# Autodesk Inventor assembly: Нога левая в сборе_MIR
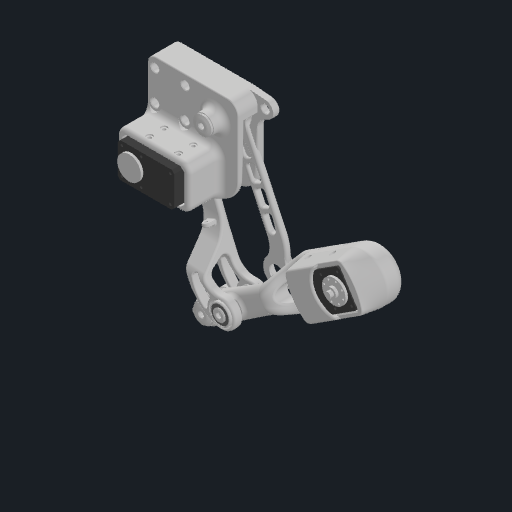
[picture p0: Inventor's stored thumbnail of the model, 512x512]
Saved by Autodesk Inventor 2025 (Build 290162010, 162A)
## iProperties
Created: 2024-06-21
Part Number: Нога левая в сборе_MIR
Document SubType Name: Assembly
Designer: Edward_Higgins
Author: Edward_Higgins
## Documents named in this file (16)
- D:\Users\Edward_Higgins\Desktop\ZAVOD\Робот Сколково\Нога левая в сборе_MIR.iam
- D:\Users\Edward_Higgins\Desktop\ZAVOD\Робот Сколково\Тяга передняя_MIR.ipt
- D:\Users\Edward_Higgins\Desktop\ZAVOD\Робот Сколково\DYNAMIXEL XM430-W350.ipt
- D:\Users\Edward_Higgins\Desktop\ZAVOD\Робот Сколково\Корпус ноги_MIR.ipt
- D:\Users\Edward_Higgins\Desktop\ZAVOD\Робот Сколково\Голень в сборе.iam
- D:\Users\Edward_Higgins\Desktop\ZAVOD\Робот Сколково\Тяга задняя 2_MIR.ipt
- D:\Users\Edward_Higgins\Desktop\ZAVOD\Робот Сколково\Подшипник.ipt
- D:\Users\Edward_Higgins\Desktop\ZAVOD\Робот Сколково\Стопорная шайба.ipt
- D:\Users\Edward_Higgins\Desktop\ZAVOD\Робот Сколково\Шайба.ipt
- D:\Users\Edward_Higgins\Desktop\ZAVOD\Робот Сколково\Ось односторонняя.ipt
- D:\Users\Edward_Higgins\Desktop\ZAVOD\Робот Сколково\Нога левая в сборе\AIP\FEA\ew5x1yt5s.fins
- D:\Users\Edward_Higgins\Desktop\ZAVOD\Робот Сколково\Нога левая в сборе\AIP\FEA\ew5x1yt5s.fsat
- D:\Users\Edward_Higgins\Desktop\ZAVOD\Робот Сколково\Нога левая в сборе\AIP\FEA\ew5x1yt5s.ftes
- D:\Users\Edward_Higgins\Desktop\ZAVOD\Робот Сколково\Нога левая в сборе\AIP\FEA\ew5x1yt5s.fwiz
- D:\Users\Edward_Higgins\Desktop\ZAVOD\Робот Сколково\Нога левая в сборе\AIP\FEA\ew5x1yt6o.fmsh
- D:\Users\Edward_Higgins\Desktop\ZAVOD\Робот Сколково\Нога левая в сборе\AIP\FEA\ew5x1yt6p.fres
## Components (9 placed, 9 different names)
1. Тяга передняя левая:1 — Совмещение:84, Совмещение:85, Совмещение:28, Совмещение:29
2. DYNAMIXEL XM430-W350:1 — Совмещение:84, Совмещение:83, Угол:1, Совмещение:29, Совмещение:30
3. Корпус ноги левый:1 — Совмещение:83, Угол:1, Совмещение:15, Совмещение:14, Совмещение:98, Совмещение:21, Совмещение:30
4. Голень в сборе:1 [sub-assembly] — Совмещение:85, Совмещение:27, Совмещение:28, Совмещение:32
5. Тяга задняя левая:1 — Совмещение:22, Совмещение:23, Совмещение:24, Совмещение:27, Совмещение:32, Совмещение:33
6. Подшипник:1 — Совмещение:93, Совмещение:25, Совмещение:26, Совмещение:33
7. Шайба:1 — Совмещение:23, Совмещение:24
8. Ось односторонняя:1 — Совмещение:98, Совмещение:93, Совмещение:21, Совмещение:22
9. Стопорная шайба:2 — Совмещение:25, Совмещение:26
## Relationships (20: Mate 19, Angle 1)
- Совмещение:84 [Mate]: Тяга передняя левая:1 ↔ DYNAMIXEL XM430-W350:1
- Совмещение:83 [Mate]: DYNAMIXEL XM430-W350:1 ↔ Корпус ноги левый:1
- Угол:1 [Angle] (0 deg): DYNAMIXEL XM430-W350:1 ↔ Корпус ноги левый:1
- Совмещение:15 [Mate]: Корпус ноги левый:1
- Совмещение:14 [Mate]: Корпус ноги левый:1
- Совмещение:85 [Mate]: Тяга передняя левая:1 ↔ Голень в сборе:1
- Совмещение:98 [Mate]: Корпус ноги левый:1 ↔ Ось односторонняя:1
- Совмещение:93 [Mate]: Подшипник:1 ↔ Ось односторонняя:1
- Совмещение:21 [Mate]: Корпус ноги левый:1 ↔ Ось односторонняя:1
- Совмещение:22 [Mate]: Тяга задняя левая:1 ↔ Ось односторонняя:1
- Совмещение:23 [Mate]: Тяга задняя левая:1 ↔ Шайба:1
- Совмещение:24 [Mate]: Тяга задняя левая:1 ↔ Шайба:1
- Совмещение:25 [Mate]: Подшипник:1 ↔ Стопорная шайба:2
- Совмещение:26 [Mate]: Подшипник:1 ↔ Стопорная шайба:2
- Совмещение:27 [Mate]: Голень в сборе:1 ↔ Тяга задняя левая:1
- Совмещение:28 [Mate]: Тяга передняя левая:1 ↔ Голень в сборе:1
- Совмещение:29 [Mate]: Тяга передняя левая:1 ↔ DYNAMIXEL XM430-W350:1
- Совмещение:30 [Mate]: DYNAMIXEL XM430-W350:1 ↔ Корпус ноги левый:1
- Совмещение:32 [Mate]: Голень в сборе:1 ↔ Тяга задняя левая:1
- Совмещение:33 [Mate]: Тяга задняя левая:1 ↔ Подшипник:1
